# Autodesk Inventor assembly: Assembly
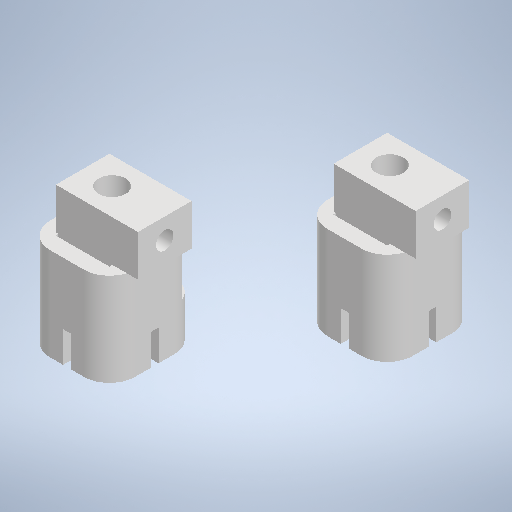
[picture p0: Inventor's stored thumbnail of the model, 512x512]
Saved by Autodesk Inventor 2025 (Build 290162010, 162A)
## iProperties
Created: 2025-02-10
Part Number: Assembly
Document SubType Name: Assembly
Designer: aduwa
Author: aduwa
## Documents named in this file (4)
- C:\Users\aduwa\OneDrive\Documents\PROJECTS\2025\CAPSTONE\V1\Assembly.iam
- C:\Users\aduwa\OneDrive\Documents\PROJECTS\2025\CAPSTONE\V1\nothced_rubik_adapter.ipt
- C:\Users\aduwa\OneDrive\Documents\PROJECTS\2025\CAPSTONE\V1\rubik_adapter.ipt
- C:\Users\aduwa\OneDrive\Documents\PROJECTS\2025\CAPSTONE\V1\motor_rubik_adapter.ipt
## Components (4 placed, 3 different names)
1. nothced_rubik_adapter:1 — Mate:1, Mate:2
2. rubik_adapter:1 — Mate:3, Mate:4
3. motor_rubik_adapter:1 — Mate:1, Mate:2
4. motor_rubik_adapter:2 — Mate:3, Mate:4
## Relationships (4: Mate 4)
- Mate:1: nothced_rubik_adapter:1 ↔ motor_rubik_adapter:1
- Mate:2: nothced_rubik_adapter:1 ↔ motor_rubik_adapter:1
- Mate:3: rubik_adapter:1 ↔ motor_rubik_adapter:2
- Mate:4: rubik_adapter:1 ↔ motor_rubik_adapter:2
